# Autodesk Inventor assembly: golfing assem
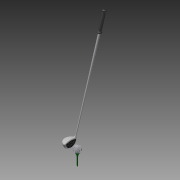
[picture p0: Inventor's stored thumbnail of the model, 180x180]
Saved by Autodesk Inventor 2014 (Build 180170000, 170)
## iProperties
Created: 2013-07-18
Part Number: golfing assem
Document SubType Name: Assembly
Designer: 5298001713
Author: 5298001713
## Documents named in this file (4)
- D:\Work\5298001713\Documents\golfing assem.iam
- R:\Student Drawings\Michael\invention (atuocad)\golf tee.ipt
- R:\Student Drawings\Michael\invention (atuocad)\golf ball.ipt
- R:\Student Drawings\Michael\invention (atuocad)\golf club.ipt
## Components (3 placed, 3 different names)
1. golf tee:1 — Flush:1, Mate:2, Flush:2, Mate:3, Mate:4
2. golf ball:1 — Flush:1, Mate:2
3. golf club:1 — Flush:2, Mate:3, Mate:4
## Relationships (5: Mate 3, Flush 2)
- Flush:1 (124.46 mm): golf tee:1 ↔ golf ball:1
- Mate:2: golf tee:1 ↔ golf ball:1
- Flush:2: golf tee:1 ↔ golf club:1
- Mate:3 (254 mm): golf tee:1 ↔ golf club:1
- Mate:4 (254 mm): golf tee:1 ↔ golf club:1
